# Autodesk Inventor assembly: strojniSklop
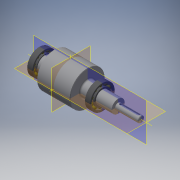
[picture p0: Inventor's stored thumbnail of the model, 180x180]
Saved by Autodesk Inventor 2018 (Build 220112000, 112)
## iProperties
Created: 2018-05-05
Part Number: strojniSklop
Document SubType Name: Assembly
Designer: Kristijan
Author: Kristijan
## Documents named in this file (3)
- C:\Users\Kristijan\Dropbox\PolitehnikaPula\4 semestar\Elementi strojeva 2\projektniZadatak\vratiloAssembly.iam
- C:\Users\Kristijan\Dropbox\PolitehnikaPula\4 semestar\Elementi strojeva 2\projektniZadatak\6209.iam
- C:\Users\Kristijan\Dropbox\PolitehnikaPula\4 semestar\Elementi strojeva 2\projektniZadatak\vratilo_kristijan.ipt
## Components (3 placed, 2 different names)
1. vratilo:1 — Mate:1, Mate:2, Mate:3, Mate:4
2. 6209:1 [sub-assembly] — Mate:1, Mate:4
3. 6209:2 [sub-assembly] — Mate:2, Mate:3
## Relationships (4: Mate 4)
- Mate:1: vratilo:1 ↔ 6209:1
- Mate:2: vratilo:1 ↔ 6209:2
- Mate:3: vratilo:1 ↔ 6209:2
- Mate:4: vratilo:1 ↔ 6209:1
